# Autodesk Inventor assembly: Foot
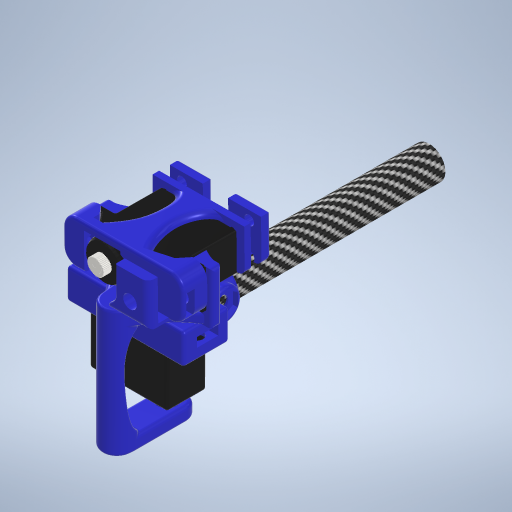
[picture p0: Inventor's stored thumbnail of the model, 512x512]
Saved by Autodesk Inventor 2023 (Build 270158000, 158)
## iProperties
Created: 2022-09-01
Part Number: Foot
Document SubType Name: Assembly
Designer: Windows10
Author: Windows10
## Documents named in this file (5)
- C:\Users\Windows10\Dropbox\Study\Climbing_Robot\CAD\new_robot_model\Foot.iam
- C:\Users\Windows10\Dropbox\Study\Climbing_Robot\CAD\new_robot_model\Carbon_Fiber_Tube_70mm.ipt
- C:\Users\Windows10\Dropbox\Study\Climbing_Robot\CAD\new_robot_model\Wrist_Servo_Holder2_v2.ipt
- C:\Users\Windows10\Dropbox\Study\Climbing_Robot\CAD\new_robot_model\adafruitMicro_servo.ipt
- C:\Users\Windows10\Dropbox\Study\Climbing_Robot\CAD\new_robot_model\Leg_Front_Rotational_Joint.ipt
## Components (4 placed, 4 different names)
1. Carbon_Fiber_Tube_70mm:1 — Mate:1
2. Wrist_Servo_Holder2_v2:1 — Mate:1, Mate:2
3. adafruitMicro_servo:1 — Mate:2, Mate:3
4. Leg_Front_Rotational_Joint:1 — Mate:3
## Relationships (3: Mate 3)
- Mate:1: Carbon_Fiber_Tube_70mm:1 ↔ Wrist_Servo_Holder2_v2:1
- Mate:2: Wrist_Servo_Holder2_v2:1 ↔ adafruitMicro_servo:1
- Mate:3: adafruitMicro_servo:1 ↔ Leg_Front_Rotational_Joint:1
